# Autodesk Inventor assembly: Intake Full Assembly
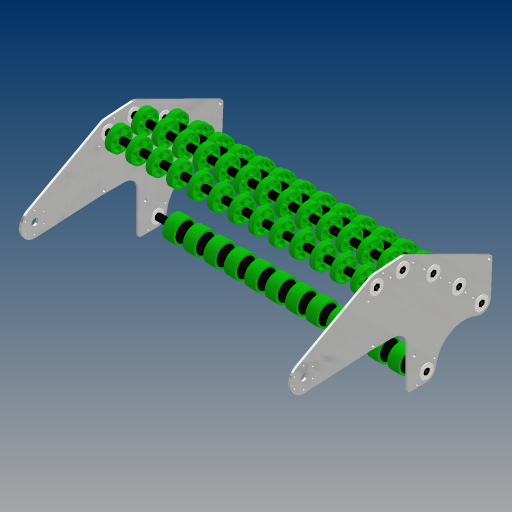
[picture p0: Inventor's stored thumbnail of the model, 512x512]
Saved by Autodesk Inventor 2024.3 (Build 283343000, 343)
## iProperties
Created: 2024-07-29
Part Number: Intake Full Assembly
Document SubType Name: Assembly
Designer: Kenji
Author: Kenji
## Documents named in this file (6)
- C:\Users\Kenji\Documents\GitHub\1622-2024-Summer-CAD-A-Thon\Intake\Intake Full Assembly.iam
- C:\Users\Kenji\Documents\GitHub\1622-2024-Summer-CAD-A-Thon\Intake\Intake Roller Plate.ipt
- C:\Users\Kenji\Documents\GitHub\1622-2024-Summer-CAD-A-Thon\COTS Library\Motion\Bearings\COTS_WCP-0783_1.125ODHexBearing.ipt
- C:\Users\Kenji\Documents\GitHub\1622-2024-Summer-CAD-A-Thon\Intake\Intake HexShaft 1.ipt
- C:\Users\Kenji\Documents\GitHub\1622-2024-Summer-CAD-A-Thon\Intake\am-3462 2IN Molded 500Hex Compliant Wheel REV2.ipt
- C:\Users\Kenji\Documents\GitHub\1622-2024-Summer-CAD-A-Thon\Intake\am-3155 2IN 500Hex Stealth Wheel REV2.iam
## Components (97 placed, 5 different names)
1. Intake Roller Plate:1 — Mate:111, Mate:112, Mate:113, Mate:114, Mate:116, Mate:117, Mate:119, Mate:120, Mate:121, Mate:122, Mate:123, Mate:124, Mate:125
2. Intake Roller Plate:2 — Mate:116, Mate:117, Mate:118, Mate:126, Mate:127, Mate:128, Mate:129
3. COTS_WCP-0783_1.125ODHexBearing:1 — Mate:25, Mate:32, Flush:11, Mate:128, Mate:129
4. COTS_WCP-0783_1.125ODHexBearing:2 — Mate:26, Mate:27, Flush:1
5. COTS_WCP-0783_1.125ODHexBearing:3 — Mate:31, Flush:9
6. COTS_WCP-0783_1.125ODHexBearing:4 — Flush:8, Mate:126, Mate:127
7. COTS_WCP-0783_1.125ODHexBearing:5 — Flush:4, Mate:118
8. COTS_WCP-0783_1.125ODHexBearing:6 — Flush:6
9. COTS_WCP-0783_1.125ODHexBearing:7 — Flush:10, Mate:111, Mate:115, Mate:124, Mate:125
10. COTS_WCP-0783_1.125ODHexBearing:8 — Mate:30, Flush:7, Mate:122, Mate:123
11. COTS_WCP-0783_1.125ODHexBearing:9 — Mate:29, Flush:5, Mate:112, Mate:121
12. COTS_WCP-0783_1.125ODHexBearing:10 — Mate:25, Flush:12
13. COTS_WCP-0783_1.125ODHexBearing:11 — Mate:26, Flush:2, Mate:114, Mate:119
14. COTS_WCP-0783_1.125ODHexBearing:12 — Mate:28, Flush:3, Mate:33, Mate:113, Mate:120
15. Intake HexShaft 1:1 — Mate:31, Flush:9, Flush:10, Mate:85, Mate:115
16. Intake HexShaft 1:2 — Mate:32, Flush:11, Flush:12, Mate:98
17. Intake HexShaft 1:3 — Mate:30, Flush:7, Flush:8, Mate:72
18. Intake HexShaft 1:4 — Mate:29, Flush:5, Flush:6, Mate:59
19. Intake HexShaft 1:5 — Mate:28, Flush:3, Flush:4
20. Intake HexShaft 1:6 — Mate:27, Flush:1, Flush:2, Mate:105
21. am-3462 2IN Molded 500Hex Compliant Wheel REV2:66 — Mate:98
22. am-3462 2IN Molded 500Hex Compliant Wheel REV2:40 — Mate:72
23. am-3462 2IN Molded 500Hex Compliant Wheel REV2:53 — Mate:85
24. am-3462 2IN Molded 500Hex Compliant Wheel REV2:25 — Mate:59
25. am-3462 2IN Molded 500Hex Compliant Wheel REV2:24 — Mate:33
26. am-3462 2IN Molded 500Hex Compliant Wheel REV2:67
27. am-3462 2IN Molded 500Hex Compliant Wheel REV2:68
28. am-3462 2IN Molded 500Hex Compliant Wheel REV2:69
29. am-3462 2IN Molded 500Hex Compliant Wheel REV2:70
30. am-3462 2IN Molded 500Hex Compliant Wheel REV2:71
31. am-3462 2IN Molded 500Hex Compliant Wheel REV2:72
32. am-3462 2IN Molded 500Hex Compliant Wheel REV2:73
33. am-3462 2IN Molded 500Hex Compliant Wheel REV2:74
34. am-3462 2IN Molded 500Hex Compliant Wheel REV2:75
35. am-3462 2IN Molded 500Hex Compliant Wheel REV2:76
36. am-3462 2IN Molded 500Hex Compliant Wheel REV2:77
37. am-3462 2IN Molded 500Hex Compliant Wheel REV2:78
38. am-3462 2IN Molded 500Hex Compliant Wheel REV2:79
39. am-3462 2IN Molded 500Hex Compliant Wheel REV2:80
40. am-3462 2IN Molded 500Hex Compliant Wheel REV2:81
41. am-3462 2IN Molded 500Hex Compliant Wheel REV2:82
42. am-3462 2IN Molded 500Hex Compliant Wheel REV2:83
43. am-3462 2IN Molded 500Hex Compliant Wheel REV2:84
44. am-3462 2IN Molded 500Hex Compliant Wheel REV2:85
45. am-3462 2IN Molded 500Hex Compliant Wheel REV2:86
46. am-3462 2IN Molded 500Hex Compliant Wheel REV2:87
47. am-3462 2IN Molded 500Hex Compliant Wheel REV2:88
48. am-3462 2IN Molded 500Hex Compliant Wheel REV2:89
49. am-3462 2IN Molded 500Hex Compliant Wheel REV2:90
50. am-3462 2IN Molded 500Hex Compliant Wheel REV2:91
51. am-3462 2IN Molded 500Hex Compliant Wheel REV2:92
52. am-3462 2IN Molded 500Hex Compliant Wheel REV2:93
53. am-3462 2IN Molded 500Hex Compliant Wheel REV2:94
54. am-3462 2IN Molded 500Hex Compliant Wheel REV2:95
55. am-3462 2IN Molded 500Hex Compliant Wheel REV2:96
56. am-3462 2IN Molded 500Hex Compliant Wheel REV2:97
57. am-3462 2IN Molded 500Hex Compliant Wheel REV2:98
58. am-3462 2IN Molded 500Hex Compliant Wheel REV2:99
59. am-3462 2IN Molded 500Hex Compliant Wheel REV2:100
60. am-3462 2IN Molded 500Hex Compliant Wheel REV2:101
61. am-3462 2IN Molded 500Hex Compliant Wheel REV2:102
62. am-3462 2IN Molded 500Hex Compliant Wheel REV2:103
63. am-3462 2IN Molded 500Hex Compliant Wheel REV2:104
64. am-3462 2IN Molded 500Hex Compliant Wheel REV2:105
65. am-3462 2IN Molded 500Hex Compliant Wheel REV2:106
66. am-3462 2IN Molded 500Hex Compliant Wheel REV2:107
67. am-3462 2IN Molded 500Hex Compliant Wheel REV2:108
68. am-3462 2IN Molded 500Hex Compliant Wheel REV2:109
69. am-3462 2IN Molded 500Hex Compliant Wheel REV2:110
70. am-3462 2IN Molded 500Hex Compliant Wheel REV2:111
71. am-3462 2IN Molded 500Hex Compliant Wheel REV2:112
72. am-3462 2IN Molded 500Hex Compliant Wheel REV2:113
73. am-3462 2IN Molded 500Hex Compliant Wheel REV2:114
74. am-3462 2IN Molded 500Hex Compliant Wheel REV2:115
75. am-3462 2IN Molded 500Hex Compliant Wheel REV2:116
76. am-3462 2IN Molded 500Hex Compliant Wheel REV2:117
77. am-3462 2IN Molded 500Hex Compliant Wheel REV2:118
78. am-3462 2IN Molded 500Hex Compliant Wheel REV2:119
79. am-3462 2IN Molded 500Hex Compliant Wheel REV2:120
80. am-3462 2IN Molded 500Hex Compliant Wheel REV2:121
81. am-3462 2IN Molded 500Hex Compliant Wheel REV2:122
82. am-3462 2IN Molded 500Hex Compliant Wheel REV2:123
83. am-3462 2IN Molded 500Hex Compliant Wheel REV2:124
84. am-3462 2IN Molded 500Hex Compliant Wheel REV2:125
85. am-3462 2IN Molded 500Hex Compliant Wheel REV2:126
86. am-3155 2IN 500Hex Stealth Wheel REV2:7 [sub-assembly] — Mate:105
87. am-3155 2IN 500Hex Stealth Wheel REV2:8 [sub-assembly]
88. am-3155 2IN 500Hex Stealth Wheel REV2:9 [sub-assembly]
89. am-3155 2IN 500Hex Stealth Wheel REV2:10 [sub-assembly]
90. am-3155 2IN 500Hex Stealth Wheel REV2:11 [sub-assembly]
91. am-3155 2IN 500Hex Stealth Wheel REV2:12 [sub-assembly]
92. am-3155 2IN 500Hex Stealth Wheel REV2:13 [sub-assembly]
93. am-3155 2IN 500Hex Stealth Wheel REV2:14 [sub-assembly]
94. am-3155 2IN 500Hex Stealth Wheel REV2:15 [sub-assembly]
95. am-3155 2IN 500Hex Stealth Wheel REV2:16 [sub-assembly]
96. am-3155 2IN 500Hex Stealth Wheel REV2:17 [sub-assembly]
97. am-3155 2IN 500Hex Stealth Wheel REV2:18 [sub-assembly]
## Component patterns: (13 elements, first: am-3462 2IN Molded 500Hex Compliant Wheel REV2:66 + am-3462 2IN Molded 500Hex Compliant Wheel REV2:40 + am-3462 2IN Molded 500Hex Compliant Wheel REV2:53 + am-3462 2IN Molded 500Hex Compliant Wheel REV2:25 + am-3462 2IN Molded 500Hex Compliant Wheel REV2:24), (12 elements, first: am-3155 2IN 500Hex Stealth Wheel REV2:7)
## Relationships (45: Mate 33, Flush 12)
- Mate:25: COTS_WCP-0783_1.125ODHexBearing:1 ↔ COTS_WCP-0783_1.125ODHexBearing:10
- Mate:26: COTS_WCP-0783_1.125ODHexBearing:2 ↔ COTS_WCP-0783_1.125ODHexBearing:11
- Mate:27: COTS_WCP-0783_1.125ODHexBearing:2 ↔ Intake HexShaft 1:6
- Flush:1: COTS_WCP-0783_1.125ODHexBearing:2 ↔ Intake HexShaft 1:6
- Flush:2: COTS_WCP-0783_1.125ODHexBearing:11 ↔ Intake HexShaft 1:6
- Mate:28: COTS_WCP-0783_1.125ODHexBearing:12 ↔ Intake HexShaft 1:5
- Flush:3: COTS_WCP-0783_1.125ODHexBearing:12 ↔ Intake HexShaft 1:5
- Flush:4: COTS_WCP-0783_1.125ODHexBearing:5 ↔ Intake HexShaft 1:5
- Mate:29: COTS_WCP-0783_1.125ODHexBearing:9 ↔ Intake HexShaft 1:4
- Flush:5: COTS_WCP-0783_1.125ODHexBearing:9 ↔ Intake HexShaft 1:4
- Flush:6: COTS_WCP-0783_1.125ODHexBearing:6 ↔ Intake HexShaft 1:4
- Mate:30: COTS_WCP-0783_1.125ODHexBearing:8 ↔ Intake HexShaft 1:3
- Flush:7: COTS_WCP-0783_1.125ODHexBearing:8 ↔ Intake HexShaft 1:3
- Flush:8: COTS_WCP-0783_1.125ODHexBearing:4 ↔ Intake HexShaft 1:3
- Mate:31: COTS_WCP-0783_1.125ODHexBearing:3 ↔ Intake HexShaft 1:1
- Flush:9: COTS_WCP-0783_1.125ODHexBearing:3 ↔ Intake HexShaft 1:1
- Flush:10: COTS_WCP-0783_1.125ODHexBearing:7 ↔ Intake HexShaft 1:1
- Mate:32: COTS_WCP-0783_1.125ODHexBearing:1 ↔ Intake HexShaft 1:2
- Flush:11: COTS_WCP-0783_1.125ODHexBearing:1 ↔ Intake HexShaft 1:2
- Flush:12: COTS_WCP-0783_1.125ODHexBearing:10 ↔ Intake HexShaft 1:2
- Mate:33: COTS_WCP-0783_1.125ODHexBearing:12 ↔ am-3462 2IN Molded 500Hex Compliant Wheel REV2:24
- Mate:59: Intake HexShaft 1:4 ↔ am-3462 2IN Molded 500Hex Compliant Wheel REV2:25
- Mate:72: Intake HexShaft 1:3 ↔ am-3462 2IN Molded 500Hex Compliant Wheel REV2:40
- Mate:85: Intake HexShaft 1:1 ↔ am-3462 2IN Molded 500Hex Compliant Wheel REV2:53
- Mate:98: Intake HexShaft 1:2 ↔ am-3462 2IN Molded 500Hex Compliant Wheel REV2:66
- Mate:105: Intake HexShaft 1:6 ↔ am-3155 2IN 500Hex Stealth Wheel REV2:7
- Mate:111: Intake Roller Plate:1 ↔ COTS_WCP-0783_1.125ODHexBearing:7
- Mate:112: Intake Roller Plate:1 ↔ COTS_WCP-0783_1.125ODHexBearing:9
- Mate:113: Intake Roller Plate:1 ↔ COTS_WCP-0783_1.125ODHexBearing:12
- Mate:114: Intake Roller Plate:1 ↔ COTS_WCP-0783_1.125ODHexBearing:11
- Mate:115: COTS_WCP-0783_1.125ODHexBearing:7 ↔ Intake HexShaft 1:1
- Mate:116: Intake Roller Plate:1 ↔ Intake Roller Plate:2
- Mate:117: Intake Roller Plate:1 ↔ Intake Roller Plate:2
- Mate:118: Intake Roller Plate:2 ↔ COTS_WCP-0783_1.125ODHexBearing:5
- Mate:119: Intake Roller Plate:1 ↔ COTS_WCP-0783_1.125ODHexBearing:11
- Mate:120: Intake Roller Plate:1 ↔ COTS_WCP-0783_1.125ODHexBearing:12
- Mate:121: Intake Roller Plate:1 ↔ COTS_WCP-0783_1.125ODHexBearing:9
- Mate:122: Intake Roller Plate:1 ↔ COTS_WCP-0783_1.125ODHexBearing:8
- Mate:123: Intake Roller Plate:1 ↔ COTS_WCP-0783_1.125ODHexBearing:8
- Mate:124: Intake Roller Plate:1 ↔ COTS_WCP-0783_1.125ODHexBearing:7
- Mate:125: Intake Roller Plate:1 ↔ COTS_WCP-0783_1.125ODHexBearing:7
- Mate:126: Intake Roller Plate:2 ↔ COTS_WCP-0783_1.125ODHexBearing:4
- Mate:127: Intake Roller Plate:2 ↔ COTS_WCP-0783_1.125ODHexBearing:4
- Mate:128: Intake Roller Plate:2 ↔ COTS_WCP-0783_1.125ODHexBearing:1
- Mate:129: Intake Roller Plate:2 ↔ COTS_WCP-0783_1.125ODHexBearing:1
